# Autodesk Inventor assembly: S2_Zaxis_500
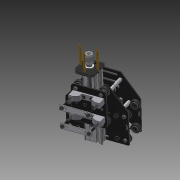
[picture p0: Inventor's stored thumbnail of the model, 180x180]
Saved by Autodesk Inventor 2014 (Build 180170000, 170)
## iProperties
Created: 2013-03-06
Part Number: S2_Zaxis_500
Document SubType Name: Assembly
Designer: Edward
Mass: 1567.3 g
Surface Area: 2632.04 cm^2
Volume: 388.503 cm^3
Density: 4.03421 g/cm^3
Author: Edward
## Documents named in this file (34)
- C:\Users\Edward\Documents\GitHub\Shapeoko_2\S2_Zaxis_500.iam
- C:\Users\Edward\Documents\GitHub\Shapeoko_2\25142-07.ipt
- C:\Users\Edward\Documents\GitHub\Shapeoko_2\25287-02.ipt
- C:\Users\Edward\Documents\GitHub\Shapeoko_2\25284-02.ipt
- C:\Users\Edward\Documents\GitHub\Shapeoko_2\25287-03.ipt
- C:\Users\Edward\Documents\GitHub\Shapeoko_2\plate_assembly.iam
- C:\Users\Edward\Documents\GitHub\Shapeoko_2\26016-01.ipt
- C:\Users\Edward\Documents\GitHub\Shapeoko_2\AS38-12-80.ipt
- C:\Users\Edward\Documents\GitHub\Shapeoko_2\91290A260.ipt
- C:\Users\Edward\Documents\GitHub\Shapeoko_2\PSBS-50.ipt
- C:\Users\Edward\Documents\GitHub\Shapeoko_2\25286-01.ipt
- C:\Users\Edward\Documents\GitHub\Shapeoko_2\25772-02.ipt
- C:\Users\Edward\Documents\GitHub\Shapeoko_2\SM-H05.ipt
- C:\Users\Edward\Documents\GitHub\Shapeoko_2\90695A040.ipt
- C:\Users\Edward\Documents\GitHub\Shapeoko_2\z-mount_plates.ipt
- C:\Users\Edward\Documents\GitHub\Shapeoko_2\30169-01.ipt
- C:\Users\Edward\Documents\GitHub\Shapeoko_2\z-axis shim.ipt
- C:\Users\Edward\Documents\GitHub\Shapeoko_2\spindle_mount_plate.ipt
- C:\Users\Edward\Documents\GitHub\Shapeoko_2\492-1101-ND.ipt
- C:\Users\Edward\Documents\GitHub\Shapeoko_2\25286-02.ipt
- C:\Users\Edward\Documents\GitHub\Shapeoko_2\SM-M08.ipt
- C:\Users\Edward\Documents\GitHub\Shapeoko_2\B18033.ipt
- C:\Users\Edward\Documents\GitHub\Shapeoko_2\25203-02.iam
- C:\Users\Edward\Documents\GitHub\Shapeoko_2\25312-14.ipt
- C:\Users\Edward\Documents\GitHub\Shapeoko_2\25286-05.ipt
- C:\Users\Edward\Documents\GitHub\Shapeoko_2\SM-TM.ipt
- C:\Users\Edward\Documents\GitHub\Shapeoko_2\SM-TM2.ipt
- C:\Users\Edward\Documents\GitHub\Shapeoko_2\25285-10.ipt
- C:\Users\Edward\Documents\GitHub\Shapeoko_2\PSM5-01MM.ipt
- C:\Users\Edward\Documents\GitHub\Shapeoko_2\simple_plate_assembly_stacked.iam
- C:\Users\Edward\Documents\GitHub\Shapeoko_2\AS38-12-64.ipt
- C:\Users\Edward\Documents\GitHub\Shapeoko_2\91290A272.ipt
- C:\Users\Edward\Documents\GitHub\Shapeoko_2\91239A233.ipt
- C:\Users\Edward\Documents\GitHub\Shapeoko_2\9714K630.ipt
## Components (147 placed, 34 different names)
1. 25142-07:1 — Mate:10, Flush:11, Flush:15, Mate:23, Mate:24, Flush:17, Insert:128, Insert:129, Angle:2, Mate:49, Flush:25
2. plate_assembly:1 [sub-assembly] — Mate:10, Flush:11, Flush:15, Flush:16, Insert:218, Insert:220, Insert:233, Insert:235, Insert:238, Insert:239, Insert:241, Insert:243, Insert:245, Insert:247, Insert:249, Insert:251
3. 25772-02:1
4. z-mount_plates:1 — Mate:25, Mate:26, Mate:28, Flush:17, Insert:115, Insert:116, Insert:117, Mate:32, Flush:18, Mate:47, Mate:48
5. z-mount_plates:2 — Insert:108, Mate:28, Insert:131, Insert:132, Insert:133
6. 30169-01:1 — Insert:108, Mate:25, Mate:26, Insert:109, Insert:110, Mate:53
7. 90695A040:1 — Insert:109
8. 90695A040:2 — Insert:110
9. 25287-03:2 — Insert:115, Insert:188
10. 25287-03:3 — Insert:116, Insert:187
11. 25287-03:4 — Insert:117, Insert:186
12. z-axis shim:1 — Insert:128, Insert:129, Mate:32, Insert:136, Insert:137, Flush:18
13. SM-H05:2 — Mate:33
14. spindle_mount_plate:1 — Insert:140, Insert:141, Insert:152, Angle:2, Mate:37, Insert:153, Insert:156, Insert:158, Insert:159, Insert:160, Insert:161, Insert:165, Insert:166, Mate:39, Insert:172, Mate:42, Insert:181, Insert:194, Insert:195, Mate:49, Flush:25
15. PSM3-01 — Insert:133, Insert:191
16. 492-1101-ND:4 — Insert:132, Insert:192
17. 492-1101-ND:5 — Insert:131, Insert:193
18. 91239A233:9 — Insert:134
19. 25287-02:36 — Insert:134, Insert:136
20. 91239A233:8 — Insert:135
21. 25287-02:37 — Insert:135, Insert:137
22. SM-M08:1 — Insert:140, Insert:141, Mate:33
23. B18033:4 — Insert:152, Mate:38
24. 25287-02:45 — Insert:156, Insert:157
25. 25203-02:7 [sub-assembly] — Mate:37, Insert:154, Insert:155
26. 25284-02:13 — Insert:157
27. 25312-14:1 — Insert:153, Insert:154
28. 25286-05:1 — Insert:155
29. SM-TM:1 — Insert:158, Insert:159, Insert:179, Mate:50, Flush:26, Flush:27, Insert:197
30. SM-TM:2 — Insert:160, Insert:161, Mate:51, Flush:28, Flush:29, Mate:52
31. 25287-02:48 — Insert:166
32. 25203-02:8 [sub-assembly]
33. 25284-02:15
34. 25312-14:2 — Insert:165
35. 25286-05:2
36. 25203-02:9 [sub-assembly]
37. 25312-14:3 — Mate:38, Mate:39
38. 25286-05:3
39. B18033:5 — Insert:172, Mate:41
40. 25203-02:10 [sub-assembly]
41. 25312-14:4 — Mate:41, Mate:42
42. 25286-05:4
43. PSM5-01MM:1 — Mate:47, Insert:189
44. PSM5-01MM:2 — Mate:48, Insert:190
45. PSBS-50:9
46. PSBS-50:11
47. PSBS-50:12
48. 25285-10:1 — Insert:188
49. 25285-10:2 — Insert:187
50. 25285-10:3 — Insert:186
51. PSM5-01MM:3 — Insert:189
52. PSM5-01MM:4 — Insert:190
53. 492-1101-ND:6 — Insert:191
54. 492-1101-ND:7 — Insert:192
55. 492-1101-ND:8 — Insert:193
56. 25286-02:10 — Insert:194
57. 25286-02:11 — Insert:195
58. SM-TM2:3 — Mate:50, Flush:26, Flush:27, Mate:51
59. SM-TM2:4 — Flush:28, Flush:29, Mate:52
60. simple_plate_assembly_stacked:1 [sub-assembly] — Insert:201, Insert:204, Insert:207, Insert:210, Insert:212, Insert:214, Insert:215, Insert:216, Insert:221, Insert:223, Insert:225, Insert:227, Insert:229, Insert:231, Insert:253
61. AS38-12-64:1 — Insert:219, Insert:220
62. 91290A272:6 — Insert:217
63. 91239A233:1 — Insert:199
64. 25203-02:12 [sub-assembly] — Insert:199, Insert:200
65. 25287-02:68 — Insert:200, Insert:201
66. 25284-02:23 — Insert:222
67. 25284-02:24 — Insert:211
68. 25287-02:71 — Insert:217, Insert:218
69. 25284-02:26 — Insert:213
70. 25287-02:72 — Insert:222, Insert:223
71. 25287-02:73 — Insert:213, Insert:214
72. 25287-02:74 — Insert:211, Insert:212
73. B18033:6 — Insert:215
74. B18033:7 — Insert:216
75. 91239A233:5
76. 25203-02:15 [sub-assembly]
77. 25287-02:75 — Insert:204
78. 91239A233:6
79. 25203-02:16 [sub-assembly]
80. 25287-02:76 — Insert:207
81. 91239A233:7
82. 25203-02:17 [sub-assembly]
83. 25287-02:77 — Insert:210
84. AS38-12-80:1 — Insert:219, Insert:221
85. 25284-02:30
86. 25287-02:78 — Insert:225
87. 25284-02:31
88. 25287-02:79 — Insert:227
89. 25284-02:32
90. 25287-02:80 — Insert:229
91. 25284-02:33
92. 25287-02:81 — Insert:231
93. 91290A272:7
94. 25287-02:82 — Insert:233
95. 91290A272:8
96. 25287-02:83 — Insert:235
97. 91290A272:9
98. 25287-02:84 — Insert:239
99. 91290A272:10
100. 25287-02:85 — Insert:238
101. AS38-12-64:7
102. AS38-12-80:2 — Insert:241
103. AS38-12-64:8
104. AS38-12-80:3 — Insert:243
105. AS38-12-64:9
106. AS38-12-80:4 — Insert:245
107. AS38-12-64:10 — Insert:247
108. AS38-12-80:5
109. 91290A272:11
110. 25287-02:86 — Insert:249
111. AS38-12-64:11 — Insert:251
112. AS38-12-80:6
113. 25284-02:34
114. 25287-02:87 — Insert:253
115. 9714K630:1 — Mate:53
116. 26016-01:5 — Mate:23, Mate:24, Flush:16, Insert:104
117. 25287-02:35 — Insert:103, Insert:104
118. 25286-01:1 — Insert:103
119. 26016-01:6
120. 25287-02:53
121. 25286-01:2
122. 26016-01:7
123. 25287-02:54
124. 25286-01:3
125. 26016-01:8
126. 25287-02:55
127. 25286-01:4
128. 25286-02:3 — Insert:179
129. 25287-02:56 — Insert:181
130. 25284-02:16
131. 25286-02:7
132. 25287-02:57
133. 25284-02:17
134. 25286-02:8
135. 25287-02:58
136. 25284-02:18
137. 25286-02:9
138. 25287-02:59
139. 25284-02:19
140. 91290A260:7
141. 25287-02:60 — Insert:197
142. 91290A260:8
143. 25287-02:61
144. 91290A260:9
145. 25287-02:62
146. 91290A260:10
147. 25287-02:63
## Component patterns: (4 elements, first: 26016-01:5 + 25287-02:35 + 25286-01:1), (4 elements, first: 25286-02:3 + 25287-02:56 + 25284-02:16), (4 elements, first: 91290A260:7 + 25287-02:60)
## Relationships (143: Insert 109, Mate 23, Flush 10, Angle 1)
- Mate:10: 25142-07:1 ↔ plate_assembly:1
- Flush:11 (-60 mm): 25142-07:1 ↔ plate_assembly:1
- Flush:15: 25142-07:1 ↔ plate_assembly:1
- Insert:103: 25287-02:35 ↔ 25286-01:1
- Mate:23: 25142-07:1 ↔ 26016-01:5
- Mate:24 (1 mm): 25142-07:1 ↔ 26016-01:5
- Flush:16 (2.5 mm): plate_assembly:1 ↔ 26016-01:5
- Insert:104 (5.4163 mm): 26016-01:5 ↔ 25287-02:35
- Insert:108 (0.5 mm): z-mount_plates:2 ↔ 30169-01:1
- Mate:25: z-mount_plates:1 ↔ 30169-01:1
- Mate:26: z-mount_plates:1 ↔ 30169-01:1
- Mate:28: z-mount_plates:1 ↔ z-mount_plates:2
- Flush:17 (-5 mm): 25142-07:1 ↔ z-mount_plates:1
- Insert:109: 30169-01:1 ↔ 90695A040:1
- Insert:110: 30169-01:1 ↔ 90695A040:2
- Insert:115: z-mount_plates:1 ↔ 25287-03:2
- Insert:116: z-mount_plates:1 ↔ 25287-03:3
- Insert:117: z-mount_plates:1 ↔ 25287-03:4
- Insert:128: 25142-07:1 ↔ z-axis shim:1
- Insert:129: 25142-07:1 ↔ z-axis shim:1
- Mate:32: z-mount_plates:1 ↔ z-axis shim:1
- Insert:131: z-mount_plates:2 ↔ 492-1101-ND:5
- Insert:132: z-mount_plates:2 ↔ 492-1101-ND:4
- Insert:133: z-mount_plates:2 ↔ PSM3-01
- Insert:134: 91239A233:9 ↔ 25287-02:36
- Insert:135: 91239A233:8 ↔ 25287-02:37
- Insert:136 (6.8137 mm): z-axis shim:1 ↔ 25287-02:36
- Insert:137 (6.8137 mm): z-axis shim:1 ↔ 25287-02:37
- Insert:140: spindle_mount_plate:1 ↔ SM-M08:1
- Insert:141: spindle_mount_plate:1 ↔ SM-M08:1
- Mate:33: SM-H05:2 ↔ SM-M08:1
- Insert:152: spindle_mount_plate:1 ↔ B18033:4
- Angle:2 (0 deg): 25142-07:1 ↔ spindle_mount_plate:1
- Mate:37: spindle_mount_plate:1 ↔ 25203-02:7
- Insert:153: spindle_mount_plate:1 ↔ 25312-14:1
- Insert:154: 25203-02:7 ↔ 25312-14:1
- Insert:155: 25203-02:7 ↔ 25286-05:1
- Insert:156: spindle_mount_plate:1 ↔ 25287-02:45
- Insert:157: 25287-02:45 ↔ 25284-02:13
- Insert:158: spindle_mount_plate:1 ↔ SM-TM:1
- Insert:159: spindle_mount_plate:1 ↔ SM-TM:1
- Insert:160: spindle_mount_plate:1 ↔ SM-TM:2
- Insert:161: spindle_mount_plate:1 ↔ SM-TM:2
- [Insert]: 25203-02:8 ↔ 25312-14:2
- [Insert]: 25203-02:8 ↔ 25286-05:2
- [Insert]: 25287-02:48 ↔ 25284-02:15
- Insert:165: spindle_mount_plate:1 ↔ 25312-14:2
- Insert:166: spindle_mount_plate:1 ↔ 25287-02:48
- [Insert]: 25203-02:9 ↔ 25312-14:3
- [Insert]: 25203-02:9 ↔ 25286-05:3
- Mate:38: B18033:4 ↔ 25312-14:3
- Mate:39: spindle_mount_plate:1 ↔ 25312-14:3
- Flush:18 (0.598 mm): z-mount_plates:1 ↔ z-axis shim:1
- [Insert]: 25203-02:10 ↔ 25312-14:4
- [Insert]: 25203-02:10 ↔ 25286-05:4
- [Mate]: B18033:5 ↔ 25312-14:4
- Insert:172: spindle_mount_plate:1 ↔ B18033:5
- Mate:41: B18033:5 ↔ 25312-14:4
- Mate:42: spindle_mount_plate:1 ↔ 25312-14:4
- Insert:179: SM-TM:1 ↔ 25286-02:3
- [Insert]: 25287-02:56 ↔ 25284-02:16
- Insert:181: spindle_mount_plate:1 ↔ 25287-02:56
- Insert:186: 25287-03:4 ↔ 25285-10:3
- Insert:187: 25287-03:3 ↔ 25285-10:2
- Insert:188: 25287-03:2 ↔ 25285-10:1
- [Mate]: 91239A233:8 ↔ PSM5-01MM:1
- [Mate]: 91239A233:9 ↔ PSM5-01MM:2
- Mate:47: z-mount_plates:1 ↔ PSM5-01MM:1
- Mate:48: z-mount_plates:1 ↔ PSM5-01MM:2
- Insert:189: PSM5-01MM:1 ↔ PSM5-01MM:3
- Insert:190: PSM5-01MM:2 ↔ PSM5-01MM:4
- Insert:191: PSM3-01 ↔ 492-1101-ND:6
- Insert:192: 492-1101-ND:4 ↔ 492-1101-ND:7
- Insert:193: 492-1101-ND:5 ↔ 492-1101-ND:8
- Insert:194: spindle_mount_plate:1 ↔ 25286-02:10
- Insert:195: spindle_mount_plate:1 ↔ 25286-02:11
- Mate:49 (12.7 mm): 25142-07:1 ↔ spindle_mount_plate:1
- Flush:25 (-25 mm): 25142-07:1 ↔ spindle_mount_plate:1
- Mate:50 (40 mm): SM-TM:1 ↔ SM-TM2:3
- Flush:26: SM-TM:1 ↔ SM-TM2:3
- Flush:27: SM-TM:1 ↔ SM-TM2:3
- Mate:51 (40 mm): SM-TM:2 ↔ SM-TM2:3
- Flush:28: SM-TM:2 ↔ SM-TM2:4
- Flush:29: SM-TM:2 ↔ SM-TM2:4
- [Insert]: 91290A260:7 ↔ 25287-02:60
- Insert:197 (42 mm): SM-TM:1 ↔ 25287-02:60
- Mate:52 (40 mm): SM-TM:2 ↔ SM-TM2:4
- Insert:199: 91239A233:1 ↔ 25203-02:12
- Insert:200: 25203-02:12 ↔ 25287-02:68
- Insert:201: simple_plate_assembly_stacked:1 ↔ 25287-02:68
- [Insert]: 91239A233:5 ↔ 25203-02:15
- [Insert]: 25203-02:15 ↔ 25287-02:75
- Insert:204: simple_plate_assembly_stacked:1 ↔ 25287-02:75
- [Insert]: 91239A233:6 ↔ 25203-02:16
- [Insert]: 25203-02:16 ↔ 25287-02:76
- Insert:207: simple_plate_assembly_stacked:1 ↔ 25287-02:76
- [Insert]: 91239A233:7 ↔ 25203-02:17
- [Insert]: 25203-02:17 ↔ 25287-02:77
- Insert:210: simple_plate_assembly_stacked:1 ↔ 25287-02:77
- Insert:211: 25284-02:24 ↔ 25287-02:74
- Insert:212: simple_plate_assembly_stacked:1 ↔ 25287-02:74
- Insert:213: 25284-02:26 ↔ 25287-02:73
- Insert:214: simple_plate_assembly_stacked:1 ↔ 25287-02:73
- Insert:215: simple_plate_assembly_stacked:1 ↔ B18033:6
- Insert:216: simple_plate_assembly_stacked:1 ↔ B18033:7
- Insert:217: 91290A272:6 ↔ 25287-02:71
- Insert:218: plate_assembly:1 ↔ 25287-02:71
- Insert:219: AS38-12-64:1 ↔ AS38-12-80:1
- Insert:220: plate_assembly:1 ↔ AS38-12-64:1
- Insert:221: simple_plate_assembly_stacked:1 ↔ AS38-12-80:1
- Insert:222: 25284-02:23 ↔ 25287-02:72
- Insert:223: simple_plate_assembly_stacked:1 ↔ 25287-02:72
- [Insert]: 25284-02:30 ↔ 25287-02:78
- Insert:225: simple_plate_assembly_stacked:1 ↔ 25287-02:78
- [Insert]: 25284-02:31 ↔ 25287-02:79
- Insert:227: simple_plate_assembly_stacked:1 ↔ 25287-02:79
- [Insert]: 25284-02:32 ↔ 25287-02:80
- Insert:229: simple_plate_assembly_stacked:1 ↔ 25287-02:80
- [Insert]: 25284-02:33 ↔ 25287-02:81
- Insert:231: simple_plate_assembly_stacked:1 ↔ 25287-02:81
- [Insert]: 91290A272:7 ↔ 25287-02:82
- Insert:233: plate_assembly:1 ↔ 25287-02:82
- [Insert]: 91290A272:8 ↔ 25287-02:83
- Insert:235: plate_assembly:1 ↔ 25287-02:83
- [Insert]: 91290A272:9 ↔ 25287-02:84
- [Insert]: 91290A272:10 ↔ 25287-02:85
- Insert:238: plate_assembly:1 ↔ 25287-02:85
- Insert:239: plate_assembly:1 ↔ 25287-02:84
- [Insert]: AS38-12-64:7 ↔ AS38-12-80:2
- Insert:241: plate_assembly:1 ↔ AS38-12-80:2
- [Insert]: AS38-12-64:8 ↔ AS38-12-80:3
- Insert:243: plate_assembly:1 ↔ AS38-12-80:3
- [Insert]: AS38-12-64:9 ↔ AS38-12-80:4
- Insert:245: plate_assembly:1 ↔ AS38-12-80:4
- [Insert]: AS38-12-64:10 ↔ AS38-12-80:5
- Insert:247: plate_assembly:1 ↔ AS38-12-64:10
- [Insert]: 91290A272:11 ↔ 25287-02:86
- Insert:249: plate_assembly:1 ↔ 25287-02:86
- [Insert]: AS38-12-64:11 ↔ AS38-12-80:6
- Insert:251: plate_assembly:1 ↔ AS38-12-64:11
- [Insert]: 25284-02:34 ↔ 25287-02:87
- Insert:253: simple_plate_assembly_stacked:1 ↔ 25287-02:87
- Mate:53: 30169-01:1 ↔ 9714K630:1
## Named parameters: d159_d104 = 0 mm, d101_d55_d51 = 0 mm, d212_d101_d55_d51 = 0 mm, d254_d246 = 0 mm, d255_d247 = 0 mm, d256_d249 = 0 mm, d259_d246 = 0 mm, d260_d247 = 0 mm, d267_d259_d246 = 0 mm, d268_d260_d247 = 0 mm, d269_d262 = 0 mm, d293_d249 = 0 mm, d331_d137 = 0 mm, d344_d341 = 0 mm, d345_d342 = 0 mm, d347_d341 = 0 mm, d348_d342 = 0 mm, d350_d341 = 0 mm, d351_d342 = 0 mm, d366_d364 = 0 mm, d368_d364 = 0 mm, d370_d364 = 0 mm, d372_d364 = 0 mm, d374_d359 = 0 mm, d376_d359 = 0 mm, d378_d359 = 0 mm, d379_d359 = 0 mm, d382_d361 = 0 mm, d384_d361 = 0 mm, d386_d361 = 0 mm, d388_d361 = 0 mm, d390_d379_d359 = 0 mm, d392_d388_d361 = 0 mm, d394_d372_d364 = 0 mm
